# Autodesk Inventor assembly: Crossbrace
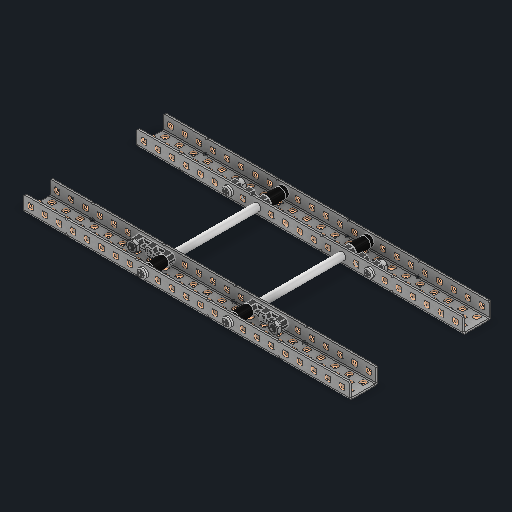
[picture p0: Inventor's stored thumbnail of the model, 512x512]
Saved by Autodesk Inventor 2025.1 (Build 291241000, 241)
## iProperties
Created: 2024-11-28
Part Number: Crossbrace
Document SubType Name: Assembly
Designer: avere
Author: avere
## Documents named in this file (10)
- C:\Users\avere\VEX\High Stakes\CAD\Codie\Chassis\Crossbrace.iam
- C:\Users\avere\VEX\High Stakes\CAD\ROBOPROS-CAD-Inventor\Structure\C Channel\Aluminum 1x2x1\Alu C 1x2x1x23.ipt
- C:\Users\avere\VEX\High Stakes\CAD\ROBOPROS-CAD-Inventor\Structure\Nylon Standoff Rounded\Nylon Standoff 3.000.ipt
- C:\Users\avere\VEX\High Stakes\CAD\ROBOPROS-CAD-Inventor\Motion\Shaft LS\Bearing Flat Low Profile.ipt
- C:\Users\avere\VEX\High Stakes\CAD\ROBOPROS-CAD-Inventor\Motion\Spacers\Spacer Nylon .375 OD\NSpacer .375 OD x .125.ipt
- C:\Users\avere\VEX\High Stakes\CAD\ROBOPROS-CAD-Inventor\Motion\Spacers\Spacer Nylon .375 OD.ipt
- C:\Users\avere\VEX\High Stakes\CAD\ROBOPROS-CAD-Inventor\Motion\Spacers\Spacer Nylon .375 OD\NSpacer .375 OD x .500.ipt
- C:\Users\avere\VEX\High Stakes\CAD\ROBOPROS-CAD-Inventor\Structure\Hardware\Screw Nylon - Pan Head\NScrew Pan Head Threaded 1.250.ipt
- C:\Users\avere\VEX\High Stakes\CAD\ROBOPROS-CAD-Inventor\Structure\Hardware\Screw Nylon - Pan Head\NScrew Pan Head Threaded .500.ipt
- C:\Users\avere\VEX\High Stakes\CAD\ROBOPROS-CAD-Inventor\Structure\Hardware\Nut Nylon Thread-Forming.ipt
## Components (28 placed, 8 different names)
1. Alu C 1x2x1x23:1 — Flush:1, Mate:1, Mate:2, Insert:1, Mate:3, Insert:4, Mate:4, Insert:5, Mate:5, Insert:7, Insert:9, Insert:10, Insert:11, Insert:12, Insert:14
2. Alu C 1x2x1x23:2 — Insert:1, Mate:3, Insert:2, Insert:3
3. Nylon Standoff 3.000:1 — Insert:3
4. Nylon Standoff 3.000:2 — Insert:2
5. Bearing Flat Low Profile:1 — Insert:4, Mate:4, Insert:13
6. Bearing Flat Low Profile:2 — Insert:5, Mate:5, Insert:15
7. NSpacer .375 OD x .125:1 — Insert:6, Insert:7
8. NSpacer .375 OD x .500:2 — Insert:6
9. NSpacer .375 OD x .125:3 — Insert:9
10. NSpacer .375 OD x .500:4
11. NScrew Pan Head Threaded 1.250:1 — Insert:10
12. NScrew Pan Head Threaded 1.250:2 — Insert:12
13. NScrew Pan Head Threaded .500:1 — Insert:11
14. Nut Nylon Thread-Forming:1 — Insert:13
15. NScrew Pan Head Threaded .500:2 — Insert:14
16. Nut Nylon Thread-Forming:2 — Insert:15
17. Bearing Flat Low Profile:3 — Insert:18
18. Bearing Flat Low Profile:4 — Insert:19
19. NSpacer .375 OD x .125:5 — Insert:16
20. NSpacer .375 OD x .500:6 — Insert:16
21. NSpacer .375 OD x .125:7 — Insert:17
22. NSpacer .375 OD x .500:8 — Insert:17
23. NScrew Pan Head Threaded 1.250:3
24. NScrew Pan Head Threaded 1.250:4
25. NScrew Pan Head Threaded .500:3
26. Nut Nylon Thread-Forming:3 — Insert:18
27. NScrew Pan Head Threaded .500:4
28. Nut Nylon Thread-Forming:4 — Insert:19
## Relationships (25: Insert 19, Mate 5, Flush 1)
- Flush:1 (-146.05 mm): Alu C 1x2x1x23:1
- Mate:1 (38.1 mm): Alu C 1x2x1x23:1
- Mate:2 (19.05 mm): Alu C 1x2x1x23:1
- Insert:1 (76.2 mm): Alu C 1x2x1x23:1 ↔ Alu C 1x2x1x23:2
- Mate:3: Alu C 1x2x1x23:1 ↔ Alu C 1x2x1x23:2
- Insert:2: Alu C 1x2x1x23:2 ↔ Nylon Standoff 3.000:2
- Insert:3: Alu C 1x2x1x23:2 ↔ Nylon Standoff 3.000:1
- Insert:4: Alu C 1x2x1x23:1 ↔ Bearing Flat Low Profile:1
- Mate:4: Alu C 1x2x1x23:1 ↔ Bearing Flat Low Profile:1
- Insert:5: Alu C 1x2x1x23:1 ↔ Bearing Flat Low Profile:2
- Mate:5: Alu C 1x2x1x23:1 ↔ Bearing Flat Low Profile:2
- Insert:6: NSpacer .375 OD x .125:1 ↔ NSpacer .375 OD x .500:2
- Insert:7: Alu C 1x2x1x23:1 ↔ NSpacer .375 OD x .125:1
- [Insert]: NSpacer .375 OD x .125:3 ↔ NSpacer .375 OD x .500:4
- Insert:9: Alu C 1x2x1x23:1 ↔ NSpacer .375 OD x .125:3
- Insert:10: Alu C 1x2x1x23:1 ↔ NScrew Pan Head Threaded 1.250:1
- Insert:11: Alu C 1x2x1x23:1 ↔ NScrew Pan Head Threaded .500:1
- Insert:12: Alu C 1x2x1x23:1 ↔ NScrew Pan Head Threaded 1.250:2
- Insert:13 (1.27 mm): Bearing Flat Low Profile:1 ↔ Nut Nylon Thread-Forming:1
- Insert:14: Alu C 1x2x1x23:1 ↔ NScrew Pan Head Threaded .500:2
- Insert:15 (1.27 mm): Bearing Flat Low Profile:2 ↔ Nut Nylon Thread-Forming:2
- Insert:16: NSpacer .375 OD x .125:5 ↔ NSpacer .375 OD x .500:6
- Insert:17: NSpacer .375 OD x .125:7 ↔ NSpacer .375 OD x .500:8
- Insert:18 (1.27 mm): Bearing Flat Low Profile:3 ↔ Nut Nylon Thread-Forming:3
- Insert:19 (1.27 mm): Bearing Flat Low Profile:4 ↔ Nut Nylon Thread-Forming:4
## Named parameters: d13_d11 = 0 mm
